# Autodesk Inventor assembly: 1.7assem
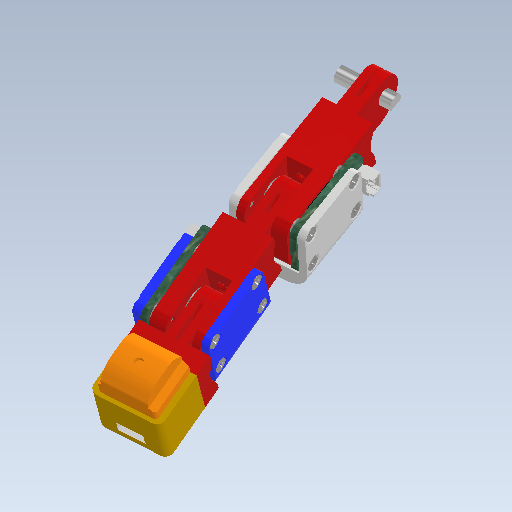
[picture p0: Inventor's stored thumbnail of the model, 512x512]
Saved by Autodesk Inventor 2020 (Build 240168000, 168)
## iProperties
Created: 2020-01-20
Part Number: 1.7assem
Document SubType Name: Assembly
Designer: sami_
Author: sami_
## Documents named in this file (4)
- C:\Users\sami_\Documents\V1.6\Workgroups\NotInProject\PINKY\finger PINKY.iam
- C:\Users\sami_\Documents\V1.6\Workgroups\NotInProject\PINKY\Fingertip assembly final.iam
- C:\Users\sami_\Documents\V1.6\LittleL1.iam
- C:\Users\sami_\Documents\V1.6\PinkyL2.iam
## Components (3 placed, 3 different names)
1. Fingertip assembly final:1 [sub-assembly]
2. LittleL1:1 [sub-assembly]
3. PinkyL2:1 [sub-assembly]
## Relationships (3: RevoluteJoint 1, WeldJoint 1, Mate 1)
- [RevoluteJoint]: LittleL1:1 ↔ PinkyL2:1
- [WeldJoint]: Fingertip assembly final:1 ↔ PinkyL2:1
- [Mate]: LittleL1:1 ↔ PinkyL2:1
